# Autodesk Inventor assembly: Body Assembly
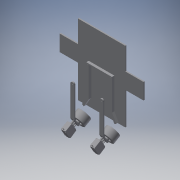
[picture p0: Inventor's stored thumbnail of the model, 180x180]
Saved by Autodesk Inventor 2019 (Build 230136000, 136)
## iProperties
Created: 2019-10-15
Part Number: Body Assembly
Document SubType Name: Assembly
Designer: User
Author: User
## Documents named in this file (4)
- C:\Robotics\CAD\2019-20_CAD\Collection\Body Assembly.iam
- C:\Robotics\CAD\2019-20_CAD\Collection\20Gen2PlatePart .ipt
- C:\Robotics\CAD\2019-20_CAD\Collection\U assembly.iam
- C:\Robotics\CAD\2019-20_CAD\Collection\U-Part Gen 2.ipt
## Components (4 placed, 3 different names)
1. 20Gen2PlatePart :1 — Mate:1, Flush:1, Flush:2, Mate:2, Mate:3, Flush:3, Flush:4, Mate:4, Mate:5
2. wheel arm assembly:1 [sub-assembly] — Mate:3, Flush:4, Mate:4
3. wheel arm assembly:2 [sub-assembly] — Mate:2, Flush:3, Mate:5
4. U-Part Gen 2:1 — Mate:1, Flush:1, Flush:2
## Relationships (9: Mate 5, Flush 4)
- Mate:1: 20Gen2PlatePart :1 ↔ U-Part Gen 2:1
- Flush:1 (-196.85 mm): 20Gen2PlatePart :1 ↔ U-Part Gen 2:1
- Flush:2 (55.88 mm): 20Gen2PlatePart :1 ↔ U-Part Gen 2:1
- Mate:2 (69.85 mm): 20Gen2PlatePart :1 ↔ wheel arm assembly:2
- Mate:3 (69.85 mm): 20Gen2PlatePart :1 ↔ wheel arm assembly:1
- Flush:3 (37.7825 mm): 20Gen2PlatePart :1 ↔ wheel arm assembly:2
- Flush:4 (-37.7825 mm): 20Gen2PlatePart :1 ↔ wheel arm assembly:1
- Mate:4 (31.75 mm): 20Gen2PlatePart :1 ↔ wheel arm assembly:1
- Mate:5 (31.75 mm): 20Gen2PlatePart :1 ↔ wheel arm assembly:2
